# Autodesk Inventor assembly: Link_03_Assembly_V02
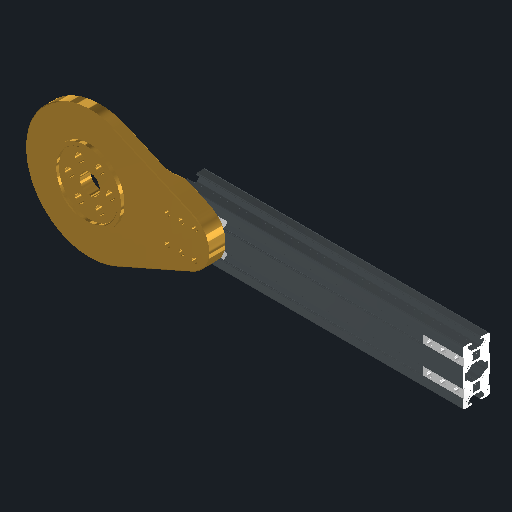
[picture p0: Inventor's stored thumbnail of the model, 512x512]
Saved by Autodesk Inventor 2026 (Build 300175000, 175)
## iProperties
Created: 2025-12-01
Part Number: Link_03_Assembly_V02
Document SubType Name: Assembly
Designer: DanielFGarzon
Mass: 268.979 g
Surface Area: 1000.75 cm^2
Volume: 146.272 cm^3
Density: 1.83889 g/cm^3
Author: DanielFGarzon
## Documents named in this file (3)
- D:\POLIMI\3RD SEMESTER\Industrial Robotics\Project\Mine\Link_03_Assembly_V02.iam
- D:\POLIMI\3RD SEMESTER\Industrial Robotics\Project\Mine\Link_03.ipt
- D:\POLIMI\3RD SEMESTER\Industrial Robotics\Project\Mine\RotationalConector_20x40_V02.ipt
## Components (2 placed, 2 different names)
1. Link_03:1 — Mate:5, Mate:6, Mate:7, Flush:1, Flush:2
2. RotationalConector_20x40_V02:1 — Mate:4, Mate:5, Mate:6, Mate:7
## Relationships (6: Mate 4, Flush 2)
- Mate:4: RotationalConector_20x40_V02:1
- Mate:5: Link_03:1 ↔ RotationalConector_20x40_V02:1
- Mate:6: Link_03:1 ↔ RotationalConector_20x40_V02:1
- Mate:7: Link_03:1 ↔ RotationalConector_20x40_V02:1
- Flush:1: Link_03:1
- Flush:2: Link_03:1
